# Autodesk Inventor assembly: Fuselage Structure Assembly
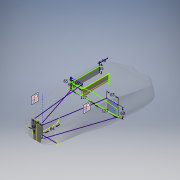
[picture p0: Inventor's stored thumbnail of the model, 180x180]
Saved by Autodesk Inventor 2018 (Build 220112000, 112)
## iProperties
Created: 2018-08-08
Part Number: Fuselage Structure Assembly
Document SubType Name: Assembly
Designer: Michael Gunderman
Author: Michael Gunderman
## Documents named in this file (7)
- C:\Users\Michael Gunderman\Documents\Special Projects\Echo 1\Echo-1-master\Echo 1\CAD work\Structures\Fuselage\Fuselage Structure Assembly.iam
- C:\Users\Michael Gunderman\Documents\Special Projects\Echo 1\Echo-1-master\Echo 1\CAD work\Preliminary Shapes\Generic Fuselage.ipt
- C:\Users\Michael Gunderman\Documents\Special Projects\Echo 1\Echo-1-master\Echo 1\CAD work\Structures\Fuselage\Fuse Structure Sketch.ipt
- C:\Users\Michael Gunderman\Documents\Special Projects\Echo 1\Echo-1-master\Echo 1\CAD work\Structures\Fuselage\Spar-Bulkhead.ipt
- C:\Users\Michael Gunderman\Documents\Special Projects\Echo 1\Echo-1-master\Echo 1\CAD work\Structures\Fuselage\Motor Mount.ipt
- C:\Users\Michael Gunderman\Documents\Special Projects\Echo 1\Echo-1-master\Echo 1\CAD work\Structures\Fuselage\Outboard wing brace.ipt
- C:\Users\Michael Gunderman\Documents\Special Projects\Echo 1\Echo-1-master\Echo 1\CAD work\Structures\Fuselage\Inboard Wing Brace.ipt
## Components (6 placed, 6 different names)
1. Generic Fuselage:1 — Mate:6
2. Fuse Structure Sketch:1 — Mate:4, Mate:5, Angle:1, Mate:8, Mate:9, Mate:10, Mate:11, Flush:3, Mate:12
3. Spar-Bulkhead:1 — Mate:2, Mate:7, Mate:8, Mate:9
4. Motor Mount:1 — Mate:4, Mate:5, Angle:1, Flush:2
5. Outboard wing brace:1 — Mate:10, Mate:11
6. Inboard Wing Brace:1 — Flush:3, Mate:12
## Relationships (13: Mate 10, Flush 2, Angle 1)
- Mate:2: Spar-Bulkhead:1
- Mate:4: Fuse Structure Sketch:1 ↔ Motor Mount:1
- Mate:5: Fuse Structure Sketch:1 ↔ Motor Mount:1
- Angle:1 (270 deg): Fuse Structure Sketch:1 ↔ Motor Mount:1
- Flush:2: Motor Mount:1
- Mate:6: Generic Fuselage:1
- Mate:7: Spar-Bulkhead:1
- Mate:8: Fuse Structure Sketch:1 ↔ Spar-Bulkhead:1
- Mate:9: Fuse Structure Sketch:1 ↔ Spar-Bulkhead:1
- Mate:10: Fuse Structure Sketch:1 ↔ Outboard wing brace:1
- Mate:11: Fuse Structure Sketch:1 ↔ Outboard wing brace:1
- Flush:3: Fuse Structure Sketch:1 ↔ Inboard Wing Brace:1
- Mate:12: Fuse Structure Sketch:1 ↔ Inboard Wing Brace:1
